# Autodesk Inventor assembly: Enclosre Assembly - L Frame
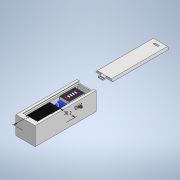
[picture p0: Inventor's stored thumbnail of the model, 180x180]
Saved by Autodesk Inventor 2022 (Build 260153000, 153)
## iProperties
Created: 2021-10-14
Part Number: Enclosre Assembly - L Frame
Document SubType Name: Assembly
Designer: tecware
Author: tecware
## Documents named in this file (7)
- C:\Users\tecware\Documents\git\calibrationKit\L-frame\components_L-frame\Enclosre Assembly - L Frame.iam
- C:\Users\tecware\Documents\git\calibrationKit\L-frame\components_L-frame\Enclosure\L Frame Enclosure.ipt
- C:\Users\tecware\Documents\git\calibrationKit\L-frame\components_L-frame\Enclosure\L Frame Enclosure Cover.ipt
- C:\Users\tecware\Documents\git\calibrationKit\components_shared\LM2596 Buck Converter.ipt
- C:\Users\tecware\Documents\git\calibrationKit\components_shared\11V 3S Lipo Battery.ipt
- C:\Users\tecware\Documents\git\calibrationKit\components_shared\SPDT Slider Switch.ipt
- C:\Users\tecware\Documents\git\calibrationKit\components_shared\Lithium Battery Capacity Indicator Module.ipt
## Components (6 placed, 6 different names)
1. L Frame Enclosure:1 — Back to back, Top, Middle
2. L Frame Enclosure Cover:1 — Back to back, Top, Middle
3. LM2596 Buck Converter:1
4. 11V 3S Lipo Battery:1
5. SPDT Slider Switch:1
6. Lithium Battery Capacity Indicator Module:1
## Relationships (3: Flush 2, Mate 1)
- Back to back [Flush]: L Frame Enclosure:1 ↔ L Frame Enclosure Cover:1
- Top [Flush]: L Frame Enclosure:1 ↔ L Frame Enclosure Cover:1
- Middle [Mate]: L Frame Enclosure:1 ↔ L Frame Enclosure Cover:1
